# Autodesk Inventor assembly: Assembly1
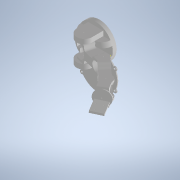
[picture p0: Inventor's stored thumbnail of the model, 180x180]
Saved by Autodesk Inventor 2022 (Build 260153000, 153)
## iProperties
Created: 2022-01-07
Part Number: Assembly1
Document SubType Name: Assembly
Designer: nguye
Author: nguye
## Documents named in this file (7)
- G:\My Drive\Study\Semester 5\Roboty Uslugowe\Project\Model\Assembly1.iam
- G:\My Drive\Study\Semester 5\Roboty Uslugowe\Project\Model\Base.ipt
- G:\My Drive\Study\Semester 5\Roboty Uslugowe\Project\Model\Baserotate.ipt
- G:\My Drive\Study\Semester 5\Roboty Uslugowe\Project\Model\Foot.ipt
- G:\My Drive\Study\Semester 5\Roboty Uslugowe\Project\Model\PartArm.ipt
- G:\My Drive\Study\Semester 5\Roboty Uslugowe\Project\Model\PartArm1.ipt
- G:\My Drive\Study\Semester 5\Roboty Uslugowe\Project\Model\gripper.ipt
## Components (8 placed, 6 different names)
1. Base:1 — Mate:1
2. Baserotate:1 — Mate:1, Mate:2, Mate:3, Mate:4, Mate:5
3. Foot:1 — Mate:2, Mate:3, Mate:6, Mate:8
4. PartArm:1 — Mate:7, Mate:8, Mate:9, Mate:10
5. Foot:2 — Mate:4, Mate:5, Mate:6, Mate:7
6. PartArm:2 — Mate:9, Mate:10, Mate:11, Mate:12
7. PartArm1:1 — Mate:11, Mate:12, Mate:13, Mate:14
8. gripper:1 — Mate:13, Mate:14
## Relationships (14: Mate 14)
- Mate:1: Base:1 ↔ Baserotate:1
- Mate:2: Baserotate:1 ↔ Foot:1
- Mate:3: Baserotate:1 ↔ Foot:1
- Mate:4: Baserotate:1 ↔ Foot:2
- Mate:5: Baserotate:1 ↔ Foot:2
- Mate:6: Foot:1 ↔ Foot:2
- Mate:7: PartArm:1 ↔ Foot:2
- Mate:8: Foot:1 ↔ PartArm:1
- Mate:9: PartArm:1 ↔ PartArm:2
- Mate:10: PartArm:1 ↔ PartArm:2
- Mate:11: PartArm:2 ↔ PartArm1:1
- Mate:12: PartArm:2 ↔ PartArm1:1
- Mate:13: PartArm1:1 ↔ gripper:1
- Mate:14: PartArm1:1 ↔ gripper:1
